# Autodesk Inventor assembly: 000-RZvector-v1
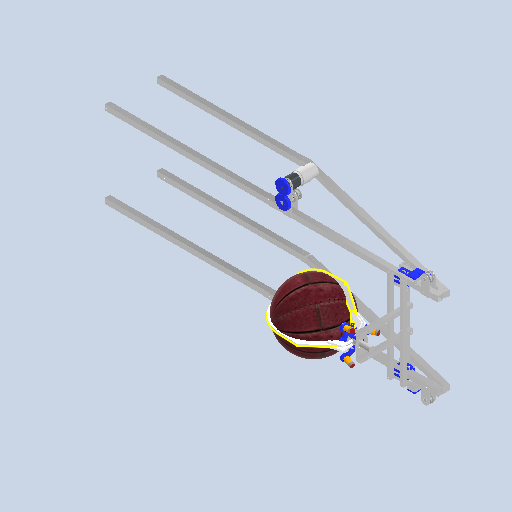
[picture p0: Inventor's stored thumbnail of the model, 512x512]
Saved by Autodesk Inventor 2025.2 (Build 292293000, 293)
## iProperties
Created: 2024-03-10
Part Number: 000-RZvector-v1
Document SubType Name: Assembly
Designer: haruy
Author: haruy
## Documents named in this file (49)
- C:\Users\haruy\Documents\ロボコン\NHK2025\cad\nagahisa\dribl\R2-Rzvector\000-RZvector-v1.iam
- C:\Users\haruy\Documents\ロボコン\NHK2025\cad\nagahisa\dribl\R2-Rzvector\RZvector-v1-ASP-Base.ipt
- C:\Users\haruy\Documents\ロボコン\NHK2025\cad\nagahisa\dribl\R2-Rzvector\RZvector-v1-Plate-E-F.ipt
- C:\Users\haruy\Documents\ロボコン\NHK2025\cad\nagahisa\dribl\R2-Rzvector\RZvector-v1-Plate-E-P-F.ipt
- C:\Users\haruy\Documents\ロボコン\NHK2025\cad\nagahisa\dribl\R2-Rzvector\encoder v2.ipt
- C:\Users\haruy\Documents\ロボコン\NHK2025\cad\nagahisa\dribl\R2-Rzvector\RZvector-v1-Plate-MM7-P-F-2.ipt
- C:\Users\haruy\Documents\ロボコン\NHK2025\cad\nagahisa\dribl\R2-Rzvector\RZvector-v1-Plate-MM7-F.ipt
- C:\Users\haruy\Documents\ロボコン\NHK2025\cad\nagahisa\dribl\R2-Rzvector\RS-775GM_004GH.iam
- C:\Users\haruy\Documents\ロボコン\NHK2025\cad\nagahisa\dribl\R2-Rzvector\000-RZvector-arm-rotate-v1.iam
- C:\Users\haruy\Documents\ロボコン\NHK2025\cad\nagahisa\dribl\R2-Rzvector\平歯車1.iam
- C:\Users\haruy\Documents\ロボコン\NHK2025\cad\nagahisa\dribl\R2-Rzvector\SCSWJ8-6.iam
- C:\Users\haruy\Documents\ロボコン\NHK2025\cad\nagahisa\dribl\R2-Rzvector\平歯車2.iam
- C:\Users\haruy\Documents\ロボコン\NHK2025\cad\nagahisa\dribl\R2-Rzvector\RZvector-v1-3DP-E-F.ipt
- C:\Users\haruy\Documents\ロボコン\NHK2025\cad\nagahisa\dribl\R2-Rzvector\TH22_bearing_12_18_19.5_sn.ipt
- C:\Users\haruy\Documents\ロボコン\NHK2025\cad\nagahisa\dribl\R2-Rzvector\平歯車3.iam
- C:\Users\haruy\Documents\ロボコン\NHK2025\cad\nagahisa\dribl\R2-Rzvector\SCSWJ12-6.iam
- C:\Users\haruy\Documents\ロボコン\NHK2025\cad\nagahisa\dribl\R2-Rzvector\MTP16XL025-A-N12.iam
- C:\Users\haruy\Documents\ロボコン\NHK2025\cad\nagahisa\dribl\R2-Rzvector\RZvector-v1-Plate-B-F.ipt
- C:\Users\haruy\Documents\ロボコン\NHK2025\cad\nagahisa\dribl\R2-Rzvector\RZvector-v1-Shaft-P-Shaft-1.ipt
- C:\Users\haruy\Documents\ロボコン\NHK2025\cad\nagahisa\dribl\R2-Rzvector\RZvector-v1-3DP-P-Spacer.ipt
- C:\Users\haruy\Documents\ロボコン\NHK2025\cad\nagahisa\dribl\R2-Rzvector\RZvector-v1-Shaft-P-Shaft-2.ipt
- C:\Users\haruy\Documents\ロボコン\NHK2025\cad\nagahisa\dribl\R2-Rzvector\RZvector-v1-Shaft-P-Shaft-3.ipt
- C:\Users\haruy\Documents\ロボコン\NHK2025\cad\nagahisa\dribl\R2-Rzvector\RZvector-v1-Shaft-P-Shaft-4.ipt
- C:\Users\haruy\Documents\ロボコン\NHK2025\cad\nagahisa\dribl\R2-Rzvector\RZvector-v1-3DP-P-Spacer-2.ipt
- C:\Users\haruy\Documents\ロボコン\NHK2025\cad\nagahisa\dribl\R2-Rzvector\RZvector-v1-3DP-P-Spacer-3.ipt
- C:\Users\haruy\Documents\ロボコン\NHK2025\cad\nagahisa\dribl\R2-Rzvector\RZvector-v1-3DP-Lm-F-under.ipt
- C:\Users\haruy\Documents\ロボコン\NHK2025\cad\nagahisa\dribl\R2-Rzvector\VX-012-1A3.iam
- C:\Users\haruy\Documents\ロボコン\NHK2025\cad\nagahisa\dribl\R2-Rzvector\RZvector-v1-Plate-P-TB-F.ipt
- C:\Users\haruy\Documents\ロボコン\NHK2025\cad\nagahisa\dribl\R2-Rzvector\RZvector-v1-Plate-MM7-P-F-3.ipt
- C:\Users\haruy\Documents\ロボコン\NHK2025\cad\nagahisa\dribl\R2-Rzvector\bear_10_15_sn.ipt
- C:\Users\haruy\Documents\ロボコン\NHK2025\cad\nagahisa\dribl\R2-Rzvector\ATP16XL025-A-N10.iam
- C:\Users\haruy\Documents\ロボコン\NHK2025\cad\nagahisa\dribl\R2-Rzvector\RZvector-v1-3DP-P-Spacer-4.ipt
- C:\Users\haruy\Documents\ロボコン\NHK2025\cad\nagahisa\dribl\R2-Rzvector\bear_f8_12_sa.ipt
- C:\Users\haruy\Documents\ロボコン\NHK2025\cad\nagahisa\dribl\R2-Rzvector\ATP16XL025-A-P8.iam
- C:\Users\haruy\Documents\ロボコン\NHK2025\cad\nagahisa\dribl\R2-Rzvector\RZvector-v1-3DP-P-Spacer-5.ipt
- C:\Users\haruy\Documents\ロボコン\NHK2025\cad\nagahisa\dribl\R2-Rzvector\平歯車5.iam
- C:\Users\haruy\Documents\ロボコン\NHK2025\cad\nagahisa\dribl\R2-Rzvector\RZvector-v1-Shaft-B-Ts.ipt
- C:\Users\haruy\Documents\ロボコン\NHK2025\cad\nagahisa\dribl\R2-Rzvector\8-19.ipt
- C:\Users\haruy\Documents\ロボコン\NHK2025\cad\nagahisa\dribl\R2-Rzvector\RZvector-v1-3DP-B-Ts-Spacer.ipt
- C:\Users\haruy\Documents\ロボコン\NHK2025\cad\nagahisa\dribl\R2-Rzvector\歯付きベルト伝達1.iam
- C:\Users\haruy\Documents\ロボコン\NHK2025\cad\nagahisa\dribl\R2-Rzvector\歯付きベルト伝達2.iam
- C:\Users\haruy\Documents\ロボコン\NHK2025\cad\nagahisa\dribl\R2-Rzvector\歯付きベルト伝達3.iam
- C:\Users\haruy\Documents\ロボコン\NHK2025\cad\nagahisa\dribl\R2-Rzvector\平歯車6.iam
- C:\Users\haruy\Documents\ロボコン\NHK2025\cad\nagahisa\dribl\R2-Rzvector\RZvector-v1-3DP-P-Spacer-6.ipt
- C:\Users\haruy\Documents\ロボコン\NHK2025\cad\nagahisa\dribl\R2-Rzvector\RZvector-v1-3DP-Lm-F-2.ipt
- C:\Users\haruy\Documents\ロボコン\NHK2025\cad\nagahisa\dribl\R2-Rzvector\RZvector-v1-MP-Tr-F.ipt
- C:\Users\haruy\Documents\ロボコン\NHK2025\cad\nagahisa\hand\grab\000-hand-grab-v3.iam
- C:\Users\haruy\Documents\ロボコン\NHK2025\cad\nagahisa\base_weel\base_weel-v1-Plate-expand-1.ipt
- C:\Users\haruy\Documents\ロボコン\NHK2025\cad\nagahisa\base_weel\base_weel-v1-Plate-expand-2.ipt
## Components (78 placed, 42 different names)
1. RZvector-v1-ASP-Base:1 — 挿入:9, 挿入:10, 挿入:11, 挿入:12, 挿入:14, 挿入:15, 挿入:26, 挿入:27, 挿入:72, 挿入:75, 挿入:104, 挿入:105, 挿入:106, 挿入:107, 挿入:120, 挿入:121, 挿入:122, 挿入:123, 挿入:155, 挿入:156, 角度:1, 角度:2, 正接:1, 正接:2, 正接:3, 挿入:182, 挿入:183, 挿入:184, 挿入:185, 挿入:186, 挿入:187, 挿入:188, 挿入:189, 挿入:190, 挿入:191, 挿入:192, 挿入:193, 挿入:194, 挿入:195, 挿入:196, 挿入:197
2. RZvector-v1-Plate-E-F:1 — 挿入:11, 挿入:12, 挿入:13, 挿入:45, 挿入:125, 挿入:128
3. RZvector-v1-Plate-E-P-F:1 — 挿入:9, 挿入:10, 挿入:46, 挿入:124, 挿入:126, 挿入:129
4. encoder v2:1 — 挿入:13, フラッシュ:4, メイト:13
5. RZvector-v1-Plate-MM7-P-F-2:2 — 挿入:14, 挿入:15, 挿入:132
6. RZvector-v1-Plate-MM7-F:1 — 挿入:26, 挿入:27, 挿入:28, 挿入:33
7. RS-775GM_004GH:1 [sub-assembly] — 挿入:28, フラッシュ:2, メイト:1
8. 000-RZvector-arm-rotate-v1:1 [sub-assembly] — 挿入:144, 挿入:145, 挿入:146, 挿入:147, 挿入:148, 挿入:149, 挿入:150, 挿入:151, 角度:2, 正接:1, 正接:2, 正接:3, 挿入:180, 挿入:181
9. 平歯車:1 [sub-assembly] — メイト:1, フラッシュ:3, 挿入:29
10. SCSWJ8-6:1 [sub-assembly] — 挿入:29
11. 平歯車:2 [sub-assembly] — 挿入:30, 挿入:31, メイト:13, メイト:14
12. RZvector-v1-3DP-E-F:1 — 挿入:30, 挿入:31
13. TH22_bearing_12_18_19.5_sn:1 — 挿入:33, メイト:4, 挿入:44, 挿入:62
14. TH22_bearing_12_18_19.5_sn:2 — 挿入:132, 挿入:135
15. 平歯車:3 [sub-assembly] — メイト:4, フラッシュ:5, 挿入:40
16. SCSWJ12-6:1 [sub-assembly] — 挿入:40
17. MTP16XL025-A-N12:3 [sub-assembly] — 挿入:44, 挿入:133
18. TH22_bearing_12_18_19.5_sn:9 — 挿入:46, 挿入:64, 挿入:67
19. TH22_bearing_12_18_19.5_sn:10 — 挿入:45, 挿入:47, 挿入:65
20. MTP16XL025-A-N12:4 [sub-assembly] — 挿入:47
21. SCSWJ12-6:3 [sub-assembly] — 挿入:163
22. MTP16XL025-A-N12:5 [sub-assembly] — 挿入:66, 挿入:142
23. RZvector-v1-Plate-B-F:1 — 挿入:146, 挿入:147, 角度:1
24. RZvector-v1-Plate-B-F:2 — 挿入:144, 挿入:145
25. RZvector-v1-Shaft-P-Shaft-1:2 — 挿入:110
26. RZvector-v1-3DP-P-Spacer:5 — 挿入:62
27. RZvector-v1-3DP-P-Spacer:6 — 挿入:133
28. RZvector-v1-3DP-P-Spacer:7 — 挿入:64
29. RZvector-v1-3DP-P-Spacer:8 — 挿入:65
30. RZvector-v1-Shaft-P-Shaft-2:1 — 挿入:66
31. RZvector-v1-Shaft-P-Shaft-3:1 — 挿入:67, メイト:15, フラッシュ:9
32. RZvector-v1-Shaft-P-Shaft-4:1 — メイト:16
33. RZvector-v1-3DP-P-Spacer-2:1 — 挿入:179
34. RZvector-v1-3DP-P-Spacer-3:2 — 挿入:135, 挿入:142
35. RZvector-v1-3DP-Lm-F-under:1 — 挿入:72, 挿入:75, 挿入:76, 挿入:77
36. VX-012-1A3:1 [sub-assembly] — 挿入:157, 挿入:158
37. VX-012-1A3:2 [sub-assembly] — 挿入:76, 挿入:77
38. RZvector-v1-Plate-P-TB-F:1 — 挿入:186, 挿入:187
39. RZvector-v1-Plate-P-TB-F:4 — 挿入:188, 挿入:189
40. RZvector-v1-Plate-MM7-P-F-3:1 — 挿入:104, 挿入:105, 挿入:108
41. RZvector-v1-Plate-MM7-P-F-3:2 — 挿入:106, 挿入:107, 挿入:109
42. bear_10_15_sn:1 — 挿入:108, 挿入:110, 挿入:111
43. bear_10_15_sn:2 — 挿入:109, 挿入:113
44. ATP16XL025-A-N10:1 [sub-assembly] — 挿入:112
45. RZvector-v1-3DP-P-Spacer-4:1 — 挿入:111, 挿入:112
46. RZvector-v1-3DP-P-Spacer-4:2 — 挿入:113
47. RZvector-v1-Shaft-P-Shaft-1:3 — 挿入:114
48. RZvector-v1-Plate-MM7-P-F-3:3 — 挿入:115, 挿入:120, 挿入:121
49. RZvector-v1-Plate-MM7-P-F-3:4 — 挿入:116, 挿入:122, 挿入:123
50. bear_10_15_sn:3 — 挿入:114, 挿入:115, 挿入:118
51. bear_10_15_sn:4 — 挿入:116, 挿入:119
52. ATP16XL025-A-N10:2 [sub-assembly] — 挿入:117, フラッシュ:7
53. RZvector-v1-3DP-P-Spacer-4:3 — 挿入:117, 挿入:118
54. RZvector-v1-3DP-P-Spacer-4:4 — 挿入:119
55. bear_f8_12_sa:1 — 挿入:124, 挿入:127
56. bear_f8_12_sa:2 — 挿入:125, 挿入:143, 挿入:179
57. ATP16XL025-A-P8:1 [sub-assembly] — 挿入:126, フラッシュ:8
58. RZvector-v1-3DP-P-Spacer-5:1 — 挿入:127
59. SCSWJ8-6:2 [sub-assembly] — 挿入:128, フラッシュ:6, 挿入:164
60. 平歯車:6 [sub-assembly] — メイト:16, メイト:17, 挿入:164
61. RZvector-v1-Shaft-B-Ts:1 — 挿入:129, 挿入:130, 挿入:131
62. 8-19:1 — 挿入:130
63. RZvector-v1-3DP-B-Ts-Spacer:1 — 挿入:131
64. 歯付きベルト伝達:1 [sub-assembly]
65. 歯付きベルト伝達:2 [sub-assembly]
66. 歯付きベルト伝達:3 [sub-assembly]
67. 平歯車:7 [sub-assembly] — メイト:15, フラッシュ:9, 挿入:163
68. RZvector-v1-3DP-P-Spacer-6:1 — 挿入:143
69. RZvector-v1-Plate-B-F:3 — 挿入:148, 挿入:149
70. RZvector-v1-Plate-B-F:4 — 挿入:150, 挿入:151
71. RZvector-v1-3DP-Lm-F-2:1 — 挿入:155, 挿入:156, 挿入:157, 挿入:158
72. RZvector-v1-MP-Tr-F:1 — 挿入:182, 挿入:183
73. RZvector-v1-MP-Tr-F:2 — 挿入:184, 挿入:185
74. 000-hand-grab-v3:1 [sub-assembly] — 挿入:180, 挿入:181
75. base_weel-v1-Plate-expand-1:1 — 挿入:196, 挿入:197
76. base_weel-v1-Plate-expand-2:1 — 挿入:194, 挿入:195
77. base_weel-v1-Plate-expand-1:2 — 挿入:190, 挿入:191
78. base_weel-v1-Plate-expand-2:2 — 挿入:192, 挿入:193
## Relationships (114: Insert 94, Flush 8, Mate 7, Tangent 3, Angle 2)
- 挿入:9 [Insert]: RZvector-v1-ASP-Base:1 ↔ RZvector-v1-Plate-E-P-F:1
- 挿入:10 [Insert]: RZvector-v1-ASP-Base:1 ↔ RZvector-v1-Plate-E-P-F:1
- 挿入:11 [Insert]: RZvector-v1-ASP-Base:1 ↔ RZvector-v1-Plate-E-F:1
- 挿入:12 [Insert]: RZvector-v1-ASP-Base:1 ↔ RZvector-v1-Plate-E-F:1
- 挿入:13 [Insert]: RZvector-v1-Plate-E-F:1 ↔ encoder v2:1
- 挿入:14 [Insert]: RZvector-v1-ASP-Base:1 ↔ RZvector-v1-Plate-MM7-P-F-2:2
- 挿入:15 [Insert]: RZvector-v1-ASP-Base:1 ↔ RZvector-v1-Plate-MM7-P-F-2:2
- 挿入:26 [Insert]: RZvector-v1-ASP-Base:1 ↔ RZvector-v1-Plate-MM7-F:1
- 挿入:27 [Insert]: RZvector-v1-ASP-Base:1 ↔ RZvector-v1-Plate-MM7-F:1
- 挿入:28 [Insert]: RZvector-v1-Plate-MM7-F:1 ↔ RS-775GM_004GH:1
- フラッシュ:2 [Flush]: RS-775GM_004GH:1
- メイト:1 [Mate]: RS-775GM_004GH:1 ↔ 平歯車:1
- フラッシュ:3 [Flush]: 平歯車:1
- 挿入:29 [Insert]: 平歯車:1 ↔ SCSWJ8-6:1
- フラッシュ:4 [Flush] (3 mm): encoder v2:1
- 挿入:30 [Insert]: 平歯車:2 ↔ RZvector-v1-3DP-E-F:1
- 挿入:31 [Insert]: 平歯車:2 ↔ RZvector-v1-3DP-E-F:1
- 挿入:33 [Insert]: RZvector-v1-Plate-MM7-F:1 ↔ TH22_bearing_12_18_19.5_sn:1
- メイト:4 [Mate]: TH22_bearing_12_18_19.5_sn:1 ↔ 平歯車:3
- フラッシュ:5 [Flush]: 平歯車:3
- 挿入:40 [Insert]: 平歯車:3 ↔ SCSWJ12-6:1
- 挿入:44 [Insert] (2.75 mm): TH22_bearing_12_18_19.5_sn:1 ↔ MTP16XL025-A-N12:3
- 挿入:45 [Insert]: RZvector-v1-Plate-E-F:1 ↔ TH22_bearing_12_18_19.5_sn:10
- 挿入:46 [Insert]: RZvector-v1-Plate-E-P-F:1 ↔ TH22_bearing_12_18_19.5_sn:9
- 挿入:47 [Insert] (2.75 mm): TH22_bearing_12_18_19.5_sn:10 ↔ MTP16XL025-A-N12:4
- 挿入:62 [Insert]: TH22_bearing_12_18_19.5_sn:1 ↔ RZvector-v1-3DP-P-Spacer:5
- 挿入:64 [Insert]: TH22_bearing_12_18_19.5_sn:9 ↔ RZvector-v1-3DP-P-Spacer:7
- 挿入:65 [Insert]: TH22_bearing_12_18_19.5_sn:10 ↔ RZvector-v1-3DP-P-Spacer:8
- 挿入:66 [Insert]: MTP16XL025-A-N12:5 ↔ RZvector-v1-Shaft-P-Shaft-2:1
- 挿入:67 [Insert]: TH22_bearing_12_18_19.5_sn:9 ↔ RZvector-v1-Shaft-P-Shaft-3:1
- 挿入:72 [Insert]: RZvector-v1-ASP-Base:1 ↔ RZvector-v1-3DP-Lm-F-under:1
- 挿入:75 [Insert]: RZvector-v1-ASP-Base:1 ↔ RZvector-v1-3DP-Lm-F-under:1
- 挿入:76 [Insert]: RZvector-v1-3DP-Lm-F-under:1 ↔ VX-012-1A3:2
- 挿入:77 [Insert]: RZvector-v1-3DP-Lm-F-under:1 ↔ VX-012-1A3:2
- 挿入:104 [Insert]: RZvector-v1-ASP-Base:1 ↔ RZvector-v1-Plate-MM7-P-F-3:1
- 挿入:105 [Insert]: RZvector-v1-ASP-Base:1 ↔ RZvector-v1-Plate-MM7-P-F-3:1
- 挿入:106 [Insert]: RZvector-v1-ASP-Base:1 ↔ RZvector-v1-Plate-MM7-P-F-3:2
- 挿入:107 [Insert]: RZvector-v1-ASP-Base:1 ↔ RZvector-v1-Plate-MM7-P-F-3:2
- 挿入:108 [Insert]: RZvector-v1-Plate-MM7-P-F-3:1 ↔ bear_10_15_sn:1
- 挿入:109 [Insert]: RZvector-v1-Plate-MM7-P-F-3:2 ↔ bear_10_15_sn:2
- 挿入:110 [Insert]: RZvector-v1-Shaft-P-Shaft-1:2 ↔ bear_10_15_sn:1
- 挿入:111 [Insert]: bear_10_15_sn:1 ↔ RZvector-v1-3DP-P-Spacer-4:1
- 挿入:112 [Insert]: ATP16XL025-A-N10:1 ↔ RZvector-v1-3DP-P-Spacer-4:1
- 挿入:113 [Insert]: bear_10_15_sn:2 ↔ RZvector-v1-3DP-P-Spacer-4:2
- 挿入:114 [Insert]: RZvector-v1-Shaft-P-Shaft-1:3 ↔ bear_10_15_sn:3
- 挿入:115 [Insert]: RZvector-v1-Plate-MM7-P-F-3:3 ↔ bear_10_15_sn:3
- 挿入:116 [Insert]: RZvector-v1-Plate-MM7-P-F-3:4 ↔ bear_10_15_sn:4
- 挿入:117 [Insert]: ATP16XL025-A-N10:2 ↔ RZvector-v1-3DP-P-Spacer-4:3
- 挿入:118 [Insert]: bear_10_15_sn:3 ↔ RZvector-v1-3DP-P-Spacer-4:3
- 挿入:119 [Insert]: bear_10_15_sn:4 ↔ RZvector-v1-3DP-P-Spacer-4:4
- 挿入:120 [Insert]: RZvector-v1-ASP-Base:1 ↔ RZvector-v1-Plate-MM7-P-F-3:3
- 挿入:121 [Insert]: RZvector-v1-ASP-Base:1 ↔ RZvector-v1-Plate-MM7-P-F-3:3
- 挿入:122 [Insert]: RZvector-v1-ASP-Base:1 ↔ RZvector-v1-Plate-MM7-P-F-3:4
- 挿入:123 [Insert]: RZvector-v1-ASP-Base:1 ↔ RZvector-v1-Plate-MM7-P-F-3:4
- 挿入:124 [Insert]: RZvector-v1-Plate-E-P-F:1 ↔ bear_f8_12_sa:1
- 挿入:125 [Insert]: RZvector-v1-Plate-E-F:1 ↔ bear_f8_12_sa:2
- 挿入:126 [Insert] (5 mm): RZvector-v1-Plate-E-P-F:1 ↔ ATP16XL025-A-P8:1
- 挿入:127 [Insert]: bear_f8_12_sa:1 ↔ RZvector-v1-3DP-P-Spacer-5:1
- 挿入:128 [Insert] (7 mm): RZvector-v1-Plate-E-F:1 ↔ SCSWJ8-6:2
- フラッシュ:6 [Flush]: SCSWJ8-6:2
- 挿入:129 [Insert]: RZvector-v1-Plate-E-P-F:1 ↔ RZvector-v1-Shaft-B-Ts:1
- 挿入:130 [Insert]: RZvector-v1-Shaft-B-Ts:1 ↔ 8-19:1
- 挿入:131 [Insert]: RZvector-v1-Shaft-B-Ts:1 ↔ RZvector-v1-3DP-B-Ts-Spacer:1
- フラッシュ:7 [Flush] (-6.25 mm): ATP16XL025-A-N10:2
- フラッシュ:8 [Flush] (-6.25 mm): ATP16XL025-A-P8:1
- 挿入:132 [Insert]: RZvector-v1-Plate-MM7-P-F-2:2 ↔ TH22_bearing_12_18_19.5_sn:2
- 挿入:133 [Insert]: MTP16XL025-A-N12:3 ↔ RZvector-v1-3DP-P-Spacer:6
- 挿入:135 [Insert]: TH22_bearing_12_18_19.5_sn:2 ↔ RZvector-v1-3DP-P-Spacer-3:2
- メイト:13 [Mate]: encoder v2:1 ↔ 平歯車:2
- メイト:14 [Mate]: 平歯車:2
- メイト:15 [Mate]: RZvector-v1-Shaft-P-Shaft-3:1 ↔ 平歯車:7
- フラッシュ:9 [Flush]: RZvector-v1-Shaft-P-Shaft-3:1 ↔ 平歯車:7
- メイト:16 [Mate]: RZvector-v1-Shaft-P-Shaft-4:1 ↔ 平歯車:6
- メイト:17 [Mate]: 平歯車:6
- 挿入:142 [Insert]: MTP16XL025-A-N12:5 ↔ RZvector-v1-3DP-P-Spacer-3:2
- 挿入:143 [Insert]: bear_f8_12_sa:2 ↔ RZvector-v1-3DP-P-Spacer-6:1
- 挿入:144 [Insert]: 000-RZvector-arm-rotate-v1:1 ↔ RZvector-v1-Plate-B-F:2
- 挿入:145 [Insert]: 000-RZvector-arm-rotate-v1:1 ↔ RZvector-v1-Plate-B-F:2
- 挿入:146 [Insert]: 000-RZvector-arm-rotate-v1:1 ↔ RZvector-v1-Plate-B-F:1
- 挿入:147 [Insert]: 000-RZvector-arm-rotate-v1:1 ↔ RZvector-v1-Plate-B-F:1
- 挿入:148 [Insert]: 000-RZvector-arm-rotate-v1:1 ↔ RZvector-v1-Plate-B-F:3
- 挿入:149 [Insert]: 000-RZvector-arm-rotate-v1:1 ↔ RZvector-v1-Plate-B-F:3
- 挿入:150 [Insert]: 000-RZvector-arm-rotate-v1:1 ↔ RZvector-v1-Plate-B-F:4
- 挿入:151 [Insert]: 000-RZvector-arm-rotate-v1:1 ↔ RZvector-v1-Plate-B-F:4
- 挿入:155 [Insert]: RZvector-v1-ASP-Base:1 ↔ RZvector-v1-3DP-Lm-F-2:1
- 挿入:156 [Insert]: RZvector-v1-ASP-Base:1 ↔ RZvector-v1-3DP-Lm-F-2:1
- 挿入:157 [Insert]: VX-012-1A3:1 ↔ RZvector-v1-3DP-Lm-F-2:1
- 挿入:158 [Insert]: VX-012-1A3:1 ↔ RZvector-v1-3DP-Lm-F-2:1
- 挿入:163 [Insert]: SCSWJ12-6:3 ↔ 平歯車:7
- 挿入:164 [Insert]: SCSWJ8-6:2 ↔ 平歯車:6
- 角度:1 [Angle] (0 deg): RZvector-v1-ASP-Base:1 ↔ RZvector-v1-Plate-B-F:1
- 角度:2 [Angle] (0 deg): RZvector-v1-ASP-Base:1 ↔ 000-RZvector-arm-rotate-v1:1
- 正接:1 [Tangent]: RZvector-v1-ASP-Base:1 ↔ 000-RZvector-arm-rotate-v1:1
- 正接:2 [Tangent]: RZvector-v1-ASP-Base:1 ↔ 000-RZvector-arm-rotate-v1:1
- 正接:3 [Tangent]: RZvector-v1-ASP-Base:1 ↔ 000-RZvector-arm-rotate-v1:1
- 挿入:179 [Insert]: RZvector-v1-3DP-P-Spacer-2:1 ↔ bear_f8_12_sa:2
- 挿入:180 [Insert]: 000-RZvector-arm-rotate-v1:1 ↔ 000-hand-grab-v3:1
- 挿入:181 [Insert]: 000-RZvector-arm-rotate-v1:1 ↔ 000-hand-grab-v3:1
- 挿入:182 [Insert]: RZvector-v1-ASP-Base:1 ↔ RZvector-v1-MP-Tr-F:1
- 挿入:183 [Insert]: RZvector-v1-ASP-Base:1 ↔ RZvector-v1-MP-Tr-F:1
- 挿入:184 [Insert]: RZvector-v1-ASP-Base:1 ↔ RZvector-v1-MP-Tr-F:2
- 挿入:185 [Insert]: RZvector-v1-ASP-Base:1 ↔ RZvector-v1-MP-Tr-F:2
- 挿入:186 [Insert]: RZvector-v1-ASP-Base:1 ↔ RZvector-v1-Plate-P-TB-F:1
- 挿入:187 [Insert]: RZvector-v1-ASP-Base:1 ↔ RZvector-v1-Plate-P-TB-F:1
- 挿入:188 [Insert]: RZvector-v1-ASP-Base:1 ↔ RZvector-v1-Plate-P-TB-F:4
- 挿入:189 [Insert]: RZvector-v1-ASP-Base:1 ↔ RZvector-v1-Plate-P-TB-F:4
- 挿入:190 [Insert]: RZvector-v1-ASP-Base:1 ↔ base_weel-v1-Plate-expand-1:2
- 挿入:191 [Insert]: RZvector-v1-ASP-Base:1 ↔ base_weel-v1-Plate-expand-1:2
- 挿入:192 [Insert]: RZvector-v1-ASP-Base:1 ↔ base_weel-v1-Plate-expand-2:2
- 挿入:193 [Insert]: RZvector-v1-ASP-Base:1 ↔ base_weel-v1-Plate-expand-2:2
- 挿入:194 [Insert]: RZvector-v1-ASP-Base:1 ↔ base_weel-v1-Plate-expand-2:1
- 挿入:195 [Insert]: RZvector-v1-ASP-Base:1 ↔ base_weel-v1-Plate-expand-2:1
- 挿入:196 [Insert]: RZvector-v1-ASP-Base:1 ↔ base_weel-v1-Plate-expand-1:1
- 挿入:197 [Insert]: RZvector-v1-ASP-Base:1 ↔ base_weel-v1-Plate-expand-1:1
